# Autodesk Inventor assembly: Payloads2
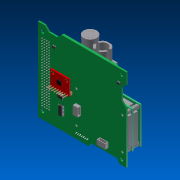
[picture p0: Inventor's stored thumbnail of the model, 180x180]
Saved by Autodesk Inventor 2012 (Build 160160000, 160)
## iProperties
Created: 2013-10-08
Part Number: Payloads2
Document SubType Name: Assembly
Designer: Thinkpad
Mass: 37.9453 g
Surface Area: 475.56 cm^2
Volume: 37.9453 cm^3
Density: 1 g/cm^3
Translation Standard: STEP AP214IS
FileName: E:\Documents and Settings\IC-Lab\Escritorio\Cubesat SUCHAI\Subsistemas\PAYLOADS\DiseÃ±o Placa\CAD\Payloads.stp
PreProcessor: Autodesk Inventor 2010
PostProcessor: Build: 160, Release: 2012 RTM - Date: Tue 03/01/2011
Sent Units: millimeter
Uncertainty: 0.01
Author: Thinkpad
## Documents named in this file (16)
- C:\Users\Thinkpad\Cubesat SUChAI\CAD\Imported Components\Payloads\Payloads2.iam
- C:\Users\Thinkpad\Cubesat SUChAI\CAD\Imported Components\Payloads\placa_pc104.ipt
- C:\Users\Thinkpad\Cubesat SUChAI\CAD\Imported Components\Payloads\530140710.ipt
- C:\Users\Thinkpad\Cubesat SUChAI\CAD\Imported Components\Payloads\961108-6804-XX.ipt
- C:\Users\Thinkpad\Cubesat SUChAI\CAD\Imported Components\Payloads\gps.ipt
- C:\Users\Thinkpad\Cubesat SUChAI\CAD\Imported Components\Payloads\placa_gyro.ipt
- C:\Users\Thinkpad\Cubesat SUChAI\CAD\Imported Components\Payloads\SOT-23-5.ipt
- C:\Users\Thinkpad\Cubesat SUChAI\CAD\Imported Components\Payloads\SOIC16 3-9mm Body Pitch 1-27mm JEDEC MS-012 AC ISSUE F.iam
- C:\Users\Thinkpad\Cubesat SUChAI\CAD\Imported Components\Payloads\SO-8.ipt
- C:\Users\Thinkpad\Cubesat SUChAI\CAD\Imported Components\Payloads\separador.ipt
- C:\Users\Thinkpad\Cubesat SUChAI\CAD\Imported Components\Payloads\pin_header_awl254-dg-g52d.ipt
- C:\Users\Thinkpad\Cubesat SUChAI\CAD\Imported Components\Payloads\Separador2.ipt
- C:\Users\Thinkpad\Cubesat SUChAI\CAD\Imported Components\Payloads\adapgps.ipt
- C:\Users\Thinkpad\Cubesat SUChAI\CAD\Imported Components\Payloads\conector_hirosedf13.ipt
- C:\Users\Thinkpad\Cubesat SUChAI\CAD\Imported Components\CAM+ADAPT\CAM+ADAPT.iam
- C:\Users\Thinkpad\Cubesat SUChAI\CAD\Imported Components\Lanzamiento LP v5\Lanzamiento LP v5.ipt
## Components (34 placed, 15 different names)
1. placa_pc104:1 — Mate:3, Flush:1, Flush:2
2. 530140710:1
3. 961108-6804-XX:1
4. gps:1
5. placa_gyro:1
6. SOT-23-5:1
7. SOT-23-5:2
8. SOT-23-5:3
9. SOT-23-5:4
10. SOIC16 3-9mm Body Pitch 1-27mm JEDEC MS-012 AC ISSUE F:1 [sub-assembly]
11. SO-8:1
12. SO-8:2
13. SO-8:3
14. SO-8:4
15. separador:1
16. separador:2
17. separador:3
18. separador:4
19. pin_header_awl254-dg-g52d:1
20. pin_header_awl254-dg-g52d:2
21. SO-8:5
22. SO-8:6
23. SO-8:7
24. SO-8:8
25. Separador2:1
26. Separador2:2
27. Separador2:3
28. Separador2:4
29. adapgps:1
30. conector_hirosedf13:1
31. conector_hirosedf13:2
32. conector_hirosedf13:3
33. CAM+ADAPT:1 [sub-assembly] — Mate:1, Mate:2
34. Lanzamiento LP v5:1 — Mate:1, Mate:2, Mate:3, Flush:1, Flush:2
## Relationships (5: Mate 3, Flush 2)
- Mate:1: CAM+ADAPT:1 ↔ Lanzamiento LP v5:1
- Mate:2: CAM+ADAPT:1 ↔ Lanzamiento LP v5:1
- Mate:3: placa_pc104:1 ↔ Lanzamiento LP v5:1
- Flush:1 (17.179 mm): placa_pc104:1 ↔ Lanzamiento LP v5:1
- Flush:2 (19.5 mm): placa_pc104:1 ↔ Lanzamiento LP v5:1
